# Autodesk Inventor assembly: wheel_assembly
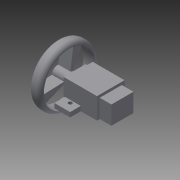
[picture p0: Inventor's stored thumbnail of the model, 180x180]
Saved by Autodesk Inventor 2015 (Build 190159000, 159)
## iProperties
Created: 2014-10-25
Part Number: wheel_assembly
Document SubType Name: Assembly
Designer: Colin
Author: Colin
## Documents named in this file (4)
- E:\Users\Colin\Documents\college\marc\MicroMouse\wheel_assembly.iam
- E:\Users\Colin\Documents\college\marc\MicroMouse\motor.ipt
- E:\Users\Colin\Documents\college\marc\MicroMouse\wheel.ipt
- E:\Users\Colin\Documents\college\marc\MicroMouse\gear_bracket.ipt
## Components (3 placed, 3 different names)
1. motor:1 — Flush:1, Flush:2, Mate:1, Insert:1
2. wheel:1 — Insert:1
3. gear_bracket:1 — Flush:1, Flush:2, Mate:1
## Relationships (4: Flush 2, Mate 1, Insert 1)
- Flush:1 (-6.35 mm): motor:1 ↔ gear_bracket:1
- Flush:2: motor:1 ↔ gear_bracket:1
- Mate:1: motor:1 ↔ gear_bracket:1
- Insert:1: motor:1 ↔ wheel:1
